# Autodesk Inventor assembly: base
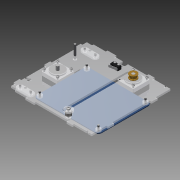
[picture p0: Inventor's stored thumbnail of the model, 180x180]
Saved by Autodesk Inventor 2013 (Build 170138000, 138)
## iProperties
Created: 2015-02-19
Part Number: base
Document SubType Name: Assembly
Designer: Noa Izumi
Author: Noa Izumi
## Documents named in this file (18)
- C:\reprap\TinyBoy_v3_20150220\assembly base.iam
- C:\reprap\TinyBoy_v3_20150220\plastic_part_04.ipt
- C:\reprap\TinyBoy_v3_20150220\stepper_28.iam
- C:\reprap\TinyBoy_v3_20150220\stepper_gear_28.ipt
- C:\reprap\TinyBoy_v3_20150220\washer_M3.ipt
- C:\reprap\TinyBoy_v3_20150220\screw_M3_16_hex.ipt
- C:\reprap\TinyBoy_v3_20150220\plastic_part_06.ipt
- C:\reprap\TinyBoy_v3_20150220\nut_M3.ipt
- C:\reprap\TinyBoy_v3_20150220\plastic_part_00.ipt
- C:\reprap\TinyBoy_v3_20150220\screw_M3_6_hex.ipt
- C:\reprap\TinyBoy_v3_20150220\switch.ipt
- C:\reprap\TinyBoy_v3_20150220\plastic_part_99.ipt
- C:\reprap\TinyBoy_v3_20150220\screw_M2_8.ipt
- C:\reprap\TinyBoy_v3_20150220\screw_M2_5_5.ipt
- C:\reprap\TinyBoy_v3_20150220\pcb_mks_1.ipt
- C:\reprap\TinyBoy_v3_20150220\screw_M3_10_hex.ipt
- C:\reprap\TinyBoy_v3_20150220\screw_M3_22_hex.ipt
- C:\reprap\TinyBoy_v3_20150220\bearing_603zz.ipt
## Components (37 placed, 17 different names)
1. stepper_28:1 [sub-assembly] — 插入:1, 插入:2, 插入:5
2. stepper_28:2 [sub-assembly] — 插入:3, 插入:4
3. plastic_part_04:1 — 插入:1, 插入:2, 插入:3, 插入:4, 插入:10, 插入:11, 插入:13, 插入:14, 插入:15, 插入:16, 插入:21, 插入:22, 插入:23, 插入:24, 插入:25, 插入:26, 插入:29, 插入:30, 插入:31, 插入:32, 插入:33, 插入:34, 插入:35, 插入:36
4. stepper_gear_28:1 — 插入:5
5. washer_M3:1 — 插入:11, 插入:12
6. washer_M3:2 — 插入:9, 插入:10
7. washer_M3:3 — 插入:7, 插入:8
8. screw_M3_16_hex:1 — 插入:6
9. bearing_603zz:1 — 插入:8, 插入:9
10. plastic_part_06:1 — 插入:6, 插入:7
11. nut_M3:1 — 插入:12
12. plastic_part_00:1 — 插入:15, 插入:16, 插入:19, 插入:20
13. plastic_part_00:2 — 插入:13, 插入:14, 插入:17, 插入:18
14. screw_M3_6_hex:1 — 插入:17
15. screw_M3_6_hex:2 — 插入:18
16. screw_M3_6_hex:3 — 插入:19
17. screw_M3_6_hex:4 — 插入:20
18. switch:1 — 插入:21, 插入:22, 插入:27, 插入:28
19. plastic_part_99:1 — 插入:23, 插入:38
20. plastic_part_99:2 — 插入:26
21. plastic_part_99:3 — 插入:25
22. plastic_part_99:4 — 插入:24, 插入:37
23. screw_M2_8:1 — 插入:27
24. screw_M2_8:2 — 插入:28
25. screw_M3_22_hex:1 — 插入:29
26. screw_M2_5_5:1 — 插入:30
27. screw_M2_5_5:2 — 插入:31
28. screw_M2_5_5:3 — 插入:32
29. screw_M2_5_5:4 — 插入:33
30. screw_M2_5_5:5 — 插入:34
31. screw_M2_5_5:6 — 插入:36
32. screw_M2_5_5:7 — 插入:35
33. pcb_mks_1:1 — 插入:37, 插入:38, 插入:39, 插入:40, 插入:41, 插入:42
34. screw_M3_10_hex:1 — 插入:42
35. screw_M3_10_hex:2 — 插入:41
36. screw_M3_10_hex:3 — 插入:40
37. screw_M3_10_hex:4 — 插入:39
## Relationships (42: Insert 42)
- 插入:1 [Insert]: stepper_28:1 ↔ plastic_part_04:1
- 插入:2 [Insert]: stepper_28:1 ↔ plastic_part_04:1
- 插入:3 [Insert]: stepper_28:2 ↔ plastic_part_04:1
- 插入:4 [Insert]: stepper_28:2 ↔ plastic_part_04:1
- 插入:5 [Insert]: stepper_28:1 ↔ stepper_gear_28:1
- 插入:6 [Insert]: screw_M3_16_hex:1 ↔ plastic_part_06:1
- 插入:7 [Insert]: washer_M3:3 ↔ plastic_part_06:1
- 插入:8 [Insert]: washer_M3:3 ↔ bearing_603zz:1
- 插入:9 [Insert]: washer_M3:2 ↔ bearing_603zz:1
- 插入:10 [Insert]: plastic_part_04:1 ↔ washer_M3:2
- 插入:11 [Insert]: plastic_part_04:1 ↔ washer_M3:1
- 插入:12 [Insert]: washer_M3:1 ↔ nut_M3:1
- 插入:13 [Insert]: plastic_part_04:1 ↔ plastic_part_00:2
- 插入:14 [Insert]: plastic_part_04:1 ↔ plastic_part_00:2
- 插入:15 [Insert]: plastic_part_04:1 ↔ plastic_part_00:1
- 插入:16 [Insert]: plastic_part_04:1 ↔ plastic_part_00:1
- 插入:17 [Insert]: plastic_part_00:2 ↔ screw_M3_6_hex:1
- 插入:18 [Insert]: plastic_part_00:2 ↔ screw_M3_6_hex:2
- 插入:19 [Insert]: plastic_part_00:1 ↔ screw_M3_6_hex:3
- 插入:20 [Insert]: plastic_part_00:1 ↔ screw_M3_6_hex:4
- 插入:21 [Insert]: plastic_part_04:1 ↔ switch:1
- 插入:22 [Insert]: plastic_part_04:1 ↔ switch:1
- 插入:23 [Insert]: plastic_part_04:1 ↔ plastic_part_99:1
- 插入:24 [Insert]: plastic_part_04:1 ↔ plastic_part_99:4
- 插入:25 [Insert]: plastic_part_04:1 ↔ plastic_part_99:3
- 插入:26 [Insert]: plastic_part_04:1 ↔ plastic_part_99:2
- 插入:27 [Insert]: switch:1 ↔ screw_M2_8:1
- 插入:28 [Insert]: switch:1 ↔ screw_M2_8:2
- 插入:29 [Insert] (2 mm): plastic_part_04:1 ↔ screw_M3_22_hex:1
- 插入:30 [Insert]: plastic_part_04:1 ↔ screw_M2_5_5:1
- 插入:31 [Insert]: plastic_part_04:1 ↔ screw_M2_5_5:2
- 插入:32 [Insert]: plastic_part_04:1 ↔ screw_M2_5_5:3
- 插入:33 [Insert]: plastic_part_04:1 ↔ screw_M2_5_5:4
- 插入:34 [Insert]: plastic_part_04:1 ↔ screw_M2_5_5:5
- 插入:35 [Insert]: plastic_part_04:1 ↔ screw_M2_5_5:7
- 插入:36 [Insert]: plastic_part_04:1 ↔ screw_M2_5_5:6
- 插入:37 [Insert]: plastic_part_99:4 ↔ pcb_mks_1:1
- 插入:38 [Insert]: plastic_part_99:1 ↔ pcb_mks_1:1
- 插入:39 [Insert]: pcb_mks_1:1 ↔ screw_M3_10_hex:4
- 插入:40 [Insert]: pcb_mks_1:1 ↔ screw_M3_10_hex:3
- 插入:41 [Insert]: pcb_mks_1:1 ↔ screw_M3_10_hex:2
- 插入:42 [Insert]: pcb_mks_1:1 ↔ screw_M3_10_hex:1
